# Autodesk Inventor assembly: lowerarms
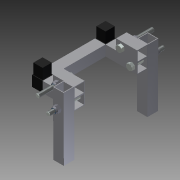
[picture p0: Inventor's stored thumbnail of the model, 180x180]
Saved by Autodesk Inventor 2011 (Build 150239000, 239)
## iProperties
Created: 2013-01-19
Part Number: lowerarms
Document SubType Name: Assembly
Designer: Danny
Author: Danny
## Documents named in this file (8)
- C:\Users\Danny\Documents\GitHub\2013CAD\2013 robot\Spiderbot\lowerarms.iam
- C:\Users\Danny\Documents\GitHub\2013CAD\2013 robot\Spiderbot\5 in 1-16.ipt
- C:\Users\Danny\Documents\GitHub\2013CAD\COTS parts\Plastic_Tubing_Connectors\3-way corner.ipt
- C:\Users\Danny\Documents\GitHub\2013CAD\2013 robot\Spiderbot\3 in 1-16.ipt
- C:\Users\Danny\Documents\GitHub\2013CAD\2013 robot\Spiderbot\short hex bolt.ipt
- C:\Users\Danny\Documents\GitHub\2013CAD\2013 robot\Spiderbot\nylock nut.ipt
- C:\Users\Danny\Documents\GitHub\2013CAD\2013 robot\Spiderbot\6 in 1-16.ipt
- C:\Users\Danny\Documents\GitHub\2013CAD\2013 robot\Spiderbot\2 in 1-16.ipt
## Components (17 placed, 7 different names)
1. 5 in 1-16:1 — Mate:1, Flush:1, Flush:2, Mate:2, Flush:3, Flush:4, Flush:7
2. 3-way corner:1 — Mate:1, Flush:1, Flush:2, Mate:3, Flush:5, Flush:6
3. 3-way corner:2 — Mate:2, Flush:3, Flush:4, Mate:4, Flush:8
4. 3 in 1-16:1 — Mate:3, Flush:5, Flush:6, Mate:5, Flush:9, Flush:10, Mate:17, Mate:18, Mate:22
5. 3 in 1-16:2 — Mate:4, Flush:7, Flush:8, Flush:11, Flush:12, Mate:6, Mate:9, Mate:10, Mate:15
6. Chassis_HexBolt_375x16x7_AndyMark_am-1055:1 — Mate:17, Mate:18, Mate:21, Mate:24
7. Chassis_HexBolt_375x16x7_AndyMark_am-1055:2 — Mate:7, Mate:8, Mate:12
8. Chassis_HexBolt_375x16x7_AndyMark_am-1055:3 — Mate:19, Mate:20, Mate:23
9. Chassis_HexBolt_375x16x7_AndyMark_am-1055:4 — Mate:9, Mate:10, Mate:11, Mate:14
10. nylock nut:1 — Mate:11, Mate:16
11. nylock nut:2 — Mate:24, Mate:26
12. nylock nut:3 — Mate:23, Mate:25
13. nylock nut:4 — Mate:12, Mate:13
14. 6 in 1-16:1 — Mate:21, Mate:22, Mate:26
15. 6 in 1-16:2 — Mate:14, Mate:15, Mate:16
16. 2 in 1-16:1 — Mate:5, Flush:9, Flush:10, Mate:19, Mate:20, Mate:25
17. 2 in 1-16:2 — Flush:11, Flush:12, Mate:6, Mate:7, Mate:8, Mate:13
## Relationships (38: Mate 26, Flush 12)
- Mate:1: 5 in 1-16:1 ↔ 3-way corner:1
- Flush:1: 5 in 1-16:1 ↔ 3-way corner:1
- Flush:2: 5 in 1-16:1 ↔ 3-way corner:1
- Mate:2: 5 in 1-16:1 ↔ 3-way corner:2
- Flush:3: 5 in 1-16:1 ↔ 3-way corner:2
- Flush:4: 5 in 1-16:1 ↔ 3-way corner:2
- Mate:3: 3-way corner:1 ↔ 3 in 1-16:1
- Flush:5: 3-way corner:1 ↔ 3 in 1-16:1
- Flush:6: 3-way corner:1 ↔ 3 in 1-16:1
- Mate:4: 3-way corner:2 ↔ 3 in 1-16:2
- Flush:7: 5 in 1-16:1 ↔ 3 in 1-16:2
- Flush:8: 3-way corner:2 ↔ 3 in 1-16:2
- Mate:5: 3 in 1-16:1 ↔ 2 in 1-16:1
- Flush:9: 3 in 1-16:1 ↔ 2 in 1-16:1
- Flush:10: 3 in 1-16:1 ↔ 2 in 1-16:1
- Flush:11: 3 in 1-16:2 ↔ 2 in 1-16:2
- Flush:12: 3 in 1-16:2 ↔ 2 in 1-16:2
- Mate:6: 3 in 1-16:2 ↔ 2 in 1-16:2
- Mate:7: Chassis_HexBolt_375x16x7_AndyMark_am-1055:2 ↔ 2 in 1-16:2
- Mate:8: Chassis_HexBolt_375x16x7_AndyMark_am-1055:2 ↔ 2 in 1-16:2
- Mate:9: 3 in 1-16:2 ↔ Chassis_HexBolt_375x16x7_AndyMark_am-1055:4
- Mate:10: 3 in 1-16:2 ↔ Chassis_HexBolt_375x16x7_AndyMark_am-1055:4
- Mate:11: Chassis_HexBolt_375x16x7_AndyMark_am-1055:4 ↔ nylock nut:1
- Mate:12: Chassis_HexBolt_375x16x7_AndyMark_am-1055:2 ↔ nylock nut:4
- Mate:13: nylock nut:4 ↔ 2 in 1-16:2
- Mate:14: Chassis_HexBolt_375x16x7_AndyMark_am-1055:4 ↔ 6 in 1-16:2
- Mate:15: 3 in 1-16:2 ↔ 6 in 1-16:2
- Mate:16: nylock nut:1 ↔ 6 in 1-16:2
- Mate:17: 3 in 1-16:1 ↔ Chassis_HexBolt_375x16x7_AndyMark_am-1055:1
- Mate:18: 3 in 1-16:1 ↔ Chassis_HexBolt_375x16x7_AndyMark_am-1055:1
- Mate:19: Chassis_HexBolt_375x16x7_AndyMark_am-1055:3 ↔ 2 in 1-16:1
- Mate:20: Chassis_HexBolt_375x16x7_AndyMark_am-1055:3 ↔ 2 in 1-16:1
- Mate:21: Chassis_HexBolt_375x16x7_AndyMark_am-1055:1 ↔ 6 in 1-16:1
- Mate:22: 3 in 1-16:1 ↔ 6 in 1-16:1
- Mate:23: Chassis_HexBolt_375x16x7_AndyMark_am-1055:3 ↔ nylock nut:3
- Mate:24: Chassis_HexBolt_375x16x7_AndyMark_am-1055:1 ↔ nylock nut:2
- Mate:25: nylock nut:3 ↔ 2 in 1-16:1
- Mate:26: nylock nut:2 ↔ 6 in 1-16:1
